# Autodesk Inventor assembly: Chassis assembly 28 Jan
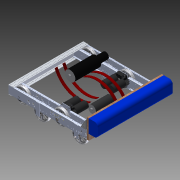
[picture p0: Inventor's stored thumbnail of the model, 180x180]
Saved by Autodesk Inventor 2014 (Build 180170000, 170)
## iProperties
Created: 2016-01-19
Part Number: Chassis assembly 28 Jan
Document SubType Name: Assembly
Designer: choices
Author: choices
## Documents named in this file (21)
- C:\Users\glasera\AppData\Local\Autodesk\Autodesk Sync\Cloud\ulanday.ian@gmail.com\2016 Robot CAD Files\ROBOT\CHASSIS\Chassis assembly 28 Jan.iam
- C:\Users\glasera\AppData\Local\Autodesk\Autodesk Sync\Cloud\ulanday.ian@gmail.com\2016 Robot CAD Files\AndyMark Chassis things\6 HiGrip with hub and double pulley.iam
- C:\Users\glasera\AppData\Local\Autodesk\Autodesk Sync\Cloud\ulanday.ian@gmail.com\2016 Robot CAD Files\AndyMark Chassis things\FR8ZZ Hex Bearing.ipt
- C:\Users\glasera\AppData\Local\Autodesk\Autodesk Sync\Cloud\ulanday.ian@gmail.com\2016 Robot CAD Files\AndyMark Chassis things\am-2598_107 2016 KOP Toughbox Mini.iam
- C:\Users\glasera\AppData\Local\Autodesk\Autodesk Sync\Cloud\ulanday.ian@gmail.com\2016 Robot CAD Files\AndyMark Chassis things\6 HiGrip with bearings, pulleys and spacers.iam
- C:\Users\glasera\AppData\Local\Autodesk\Autodesk Sync\Cloud\ulanday.ian@gmail.com\2016 Robot CAD Files\ROBOT\CHASSIS\Chass_InsideSheetTabs.ipt
- C:\Users\glasera\AppData\Local\Autodesk\Autodesk Sync\Cloud\ulanday.ian@gmail.com\2016 Robot CAD Files\AndyMark Chassis things\375-16 x 4.25 Hex Bolt_HFBOLT 0.375-16x2.5x1-C.ipt
- C:\Users\glasera\AppData\Local\Autodesk\Autodesk Sync\Cloud\ulanday.ian@gmail.com\2016 Robot CAD Files\ROBOT\CHASSIS\Chassis_OutsideSheetCustom.ipt
- C:\Users\glasera\AppData\Local\Autodesk\Autodesk Sync\Cloud\ulanday.ian@gmail.com\2016 Robot CAD Files\ROBOT\CHASSIS\Chassis_OutsideSheetCustomLeft.ipt
- C:\Users\glasera\AppData\Local\Autodesk\Autodesk Sync\Cloud\ulanday.ian@gmail.com\2016 Robot CAD Files\ROBOT\CHASSIS\Chass_InsideSheetTabsLeft.ipt
- C:\Users\glasera\AppData\Local\Autodesk\Autodesk Sync\Cloud\ulanday.ian@gmail.com\2016 Robot CAD Files\ROBOT\CHASSIS\Chass_EndCaps.ipt
- C:\Users\glasera\AppData\Local\Autodesk\Autodesk Sync\Cloud\ulanday.ian@gmail.com\2016 Robot CAD Files\ROBOT\CHASSIS\Chass_EndSheet.ipt
- C:\Users\glasera\AppData\Local\Autodesk\Autodesk Sync\Cloud\ulanday.ian@gmail.com\2016 Robot CAD Files\ROBOT\CHASSIS\Chassis_BumpermountWoodpiece.ipt
- C:\Users\glasera\AppData\Local\Autodesk\Autodesk Sync\Cloud\ulanday.ian@gmail.com\2016 Robot CAD Files\ROBOT\CHASSIS\Chassis_Bumper(29in).ipt
- C:\Users\glasera\AppData\Local\Autodesk\Autodesk Sync\Cloud\ulanday.ian@gmail.com\2016 Robot CAD Files\ROBOT\CHASSIS\Chassis_Motor.ipt
- C:\Users\glasera\AppData\Local\Autodesk\Autodesk Sync\Cloud\ulanday.ian@gmail.com\2016 Robot CAD Files\ROBOT\CHASSIS\Chassis_BumperAttachmentLeft.ipt
- C:\Users\glasera\AppData\Local\Autodesk\Autodesk Sync\Cloud\ulanday.ian@gmail.com\2016 Robot CAD Files\ROBOT\CHASSIS\Chassis_BumperAttachmentRight.ipt
- C:\Users\glasera\AppData\Local\Autodesk\Autodesk Sync\Cloud\ulanday.ian@gmail.com\2016 Robot CAD Files\ROBOT\Shooting Mechanism\Shooter_MotorTop.ipt
- C:\Users\glasera\AppData\Local\Autodesk\Autodesk Sync\Cloud\ulanday.ian@gmail.com\2016 Robot CAD Files\ROBOT\CHASSIS\Shooter_LowerMotor.ipt
- C:\Users\glasera\AppData\Local\Autodesk\Autodesk Sync\Cloud\ulanday.ian@gmail.com\2016 Robot CAD Files\ROBOT\Shooting Mechanism\Shooter_LoadingRail.ipt
- C:\Users\glasera\AppData\Local\Autodesk\Autodesk Sync\Cloud\ulanday.ian@gmail.com\2016 Robot CAD Files\ROBOT\Shooting Mechanism\Shooter_ShootingRail.ipt
## Components (35 placed, 20 different names)
1. 6 HiGrip with hub and double pulley:1 [sub-assembly] — Mate:7, Mate:8, Mate:9
2. am-2598_107 2016 KOP Toughbox Mini:1 [sub-assembly] — Mate:8, Mate:9, Mate:12, Mate:14, Flush:1, Mate:15, Mate:16, Mate:17, Insert:19, Insert:20
3. FR8ZZ Hex Bearing:1 — Mate:7, Mate:12, Mate:14, Flush:1, Mate:18, Mate:19
4. 6 HiGrip with bearings, pulleys and spacers:1 [sub-assembly] — Insert:5, Tangent:1
5. Chass_InsideSheetTabs:1 — Mate:15, Mate:16, Mate:17, Insert:5, Insert:6, Insert:8, Flush:2
6. 6 HiGrip with bearings, pulleys and spacers:2 [sub-assembly] — Insert:6
7. 6 HiGrip with bearings, pulleys and spacers:4 [sub-assembly] — Insert:8
8. Chassis_OutsideSheetCustom:1 — Mate:18, Mate:19, Insert:9, Flush:3, Mate:29, Mate:30, Flush:5, Mate:31, Mate:32, Flush:6, Angle:1, Mate:47, Mate:49
9. 375-16 x 4.25 Hex Bolt_HFBOLT 0.375-16x2.5x1-C:1 — Insert:9, Tangent:1
10. Chassis_OutsideSheetCustomLeft:1 — Insert:12, Insert:13, Insert:15, Flush:3, Mate:27, Mate:28, Flush:4, Flush:7, Flush:8, Angle:2, Angle:3
11. Chass_InsideSheetTabsLeft:1 — Mate:26, Insert:10, Insert:11, Insert:14, Insert:16, Flush:2
12. 6 HiGrip with hub and double pulley:2 [sub-assembly] — Mate:20, Mate:21, Mate:22, Mate:23
13. 6 HiGrip with bearings, pulleys and spacers:5 [sub-assembly] — Insert:13, Tangent:2
14. 6 HiGrip with bearings, pulleys and spacers:6 [sub-assembly] — Insert:15
15. 6 HiGrip with bearings, pulleys and spacers:7 [sub-assembly] — Insert:16
16. am-2598_107 2016 KOP Toughbox Mini:2 [sub-assembly] — Mate:20, Mate:21, Mate:22, Mate:24, Mate:25, Mate:26, Insert:10, Insert:11, Insert:17, Insert:18
17. FR8ZZ Hex Bearing:2 — Mate:23, Mate:24, Mate:25, Insert:12
18. 375-16 x 4.25 Hex Bolt_HFBOLT 0.375-16x2.5x1-C:2 — Insert:14, Tangent:2
19. Chass_EndCaps:1 — Mate:29, Mate:30, Flush:5, Insert:21
20. Chass_EndCaps:2 — Mate:27, Mate:28, Flush:4, Mate:33, Flush:9, Insert:22
21. Chass_EndSheet:1 — Mate:31, Mate:32, Flush:6, Flush:7
22. Chassis_BumpermountWoodpiece:1 — Mate:33, Flush:8, Flush:9, Mate:34, Flush:10, Flush:11, Mate:46
23. Chassis_Bumper(29in):1 — Mate:34, Flush:10, Flush:11
24. Chassis_Motor:1 — Insert:17
25. Chassis_Motor:2 — Insert:20
26. Chassis_Motor:3 — Insert:18, Mate:37
27. Chassis_Motor:4 — Insert:19
28. Chassis_BumperAttachmentLeft:1 — Insert:21, Angle:1
29. Chassis_BumperAttachmentRight:1 — Insert:22, Angle:2
30. Shooter_MotorTop:1 — Angle:3, Mate:37, Mate:48, Mate:49, Flush:13, Mate:50, Flush:16
31. Shooter_LowerMotor:1 — Mate:43, Mate:44, Mate:46, Mate:47, Mate:48, Flush:13
32. Shooter_LoadingRail:1 — Mate:43, Mate:45, Flush:12
33. Shooter_LoadingRail:2 — Mate:44, Mate:45, Flush:12, Flush:15
34. Shooter_ShootingRail:1 — Insert:23, Flush:14, Flush:15, Flush:16
35. Shooter_ShootingRail:2 — Insert:23, Flush:14, Mate:50
## Relationships (73: Mate 34, Insert 18, Flush 16, Angle 3, Tangent 2)
- Mate:7: 6 HiGrip with hub and double pulley:1 ↔ FR8ZZ Hex Bearing:1
- Mate:8: 6 HiGrip with hub and double pulley:1 ↔ am-2598_107 2016 KOP Toughbox Mini:1
- Mate:9: 6 HiGrip with hub and double pulley:1 ↔ am-2598_107 2016 KOP Toughbox Mini:1
- Mate:12: am-2598_107 2016 KOP Toughbox Mini:1 ↔ FR8ZZ Hex Bearing:1
- Mate:14: am-2598_107 2016 KOP Toughbox Mini:1 ↔ FR8ZZ Hex Bearing:1
- Flush:1: am-2598_107 2016 KOP Toughbox Mini:1 ↔ FR8ZZ Hex Bearing:1
- Mate:15: am-2598_107 2016 KOP Toughbox Mini:1 ↔ Chass_InsideSheetTabs:1
- Mate:16: am-2598_107 2016 KOP Toughbox Mini:1 ↔ Chass_InsideSheetTabs:1
- Mate:17: am-2598_107 2016 KOP Toughbox Mini:1 ↔ Chass_InsideSheetTabs:1
- Insert:5: 6 HiGrip with bearings, pulleys and spacers:1 ↔ Chass_InsideSheetTabs:1
- Insert:6: Chass_InsideSheetTabs:1 ↔ 6 HiGrip with bearings, pulleys and spacers:2
- Insert:8: Chass_InsideSheetTabs:1 ↔ 6 HiGrip with bearings, pulleys and spacers:4
- Mate:18: FR8ZZ Hex Bearing:1 ↔ Chassis_OutsideSheetCustom:1
- Mate:19: FR8ZZ Hex Bearing:1 ↔ Chassis_OutsideSheetCustom:1
- Insert:9: Chassis_OutsideSheetCustom:1 ↔ 375-16 x 4.25 Hex Bolt_HFBOLT 0.375-16x2.5x1-C:1
- Tangent:1: 6 HiGrip with bearings, pulleys and spacers:1 ↔ 375-16 x 4.25 Hex Bolt_HFBOLT 0.375-16x2.5x1-C:1
- Mate:20: 6 HiGrip with hub and double pulley:2 ↔ am-2598_107 2016 KOP Toughbox Mini:2
- Mate:21: 6 HiGrip with hub and double pulley:2 ↔ am-2598_107 2016 KOP Toughbox Mini:2
- Mate:22: 6 HiGrip with hub and double pulley:2 ↔ am-2598_107 2016 KOP Toughbox Mini:2
- Mate:23: 6 HiGrip with hub and double pulley:2 ↔ FR8ZZ Hex Bearing:2
- Mate:24: am-2598_107 2016 KOP Toughbox Mini:2 ↔ FR8ZZ Hex Bearing:2
- Mate:25: am-2598_107 2016 KOP Toughbox Mini:2 ↔ FR8ZZ Hex Bearing:2
- Mate:26: Chass_InsideSheetTabsLeft:1 ↔ am-2598_107 2016 KOP Toughbox Mini:2
- Insert:10: Chass_InsideSheetTabsLeft:1 ↔ am-2598_107 2016 KOP Toughbox Mini:2
- Insert:11: Chass_InsideSheetTabsLeft:1 ↔ am-2598_107 2016 KOP Toughbox Mini:2
- Insert:12: Chassis_OutsideSheetCustomLeft:1 ↔ FR8ZZ Hex Bearing:2
- Insert:13: Chassis_OutsideSheetCustomLeft:1 ↔ 6 HiGrip with bearings, pulleys and spacers:5
- Insert:14: Chass_InsideSheetTabsLeft:1 ↔ 375-16 x 4.25 Hex Bolt_HFBOLT 0.375-16x2.5x1-C:2
- Tangent:2: 6 HiGrip with bearings, pulleys and spacers:5 ↔ 375-16 x 4.25 Hex Bolt_HFBOLT 0.375-16x2.5x1-C:2
- Insert:15: Chassis_OutsideSheetCustomLeft:1 ↔ 6 HiGrip with bearings, pulleys and spacers:6
- Insert:16: Chass_InsideSheetTabsLeft:1 ↔ 6 HiGrip with bearings, pulleys and spacers:7
- Flush:2: Chass_InsideSheetTabs:1 ↔ Chass_InsideSheetTabsLeft:1
- Flush:3: Chassis_OutsideSheetCustom:1 ↔ Chassis_OutsideSheetCustomLeft:1
- Mate:27: Chassis_OutsideSheetCustomLeft:1 ↔ Chass_EndCaps:2
- Mate:28: Chassis_OutsideSheetCustomLeft:1 ↔ Chass_EndCaps:2
- Flush:4: Chassis_OutsideSheetCustomLeft:1 ↔ Chass_EndCaps:2
- Mate:29: Chassis_OutsideSheetCustom:1 ↔ Chass_EndCaps:1
- Mate:30: Chassis_OutsideSheetCustom:1 ↔ Chass_EndCaps:1
- Flush:5: Chassis_OutsideSheetCustom:1 ↔ Chass_EndCaps:1
- Mate:31: Chassis_OutsideSheetCustom:1 ↔ Chass_EndSheet:1
- Mate:32: Chassis_OutsideSheetCustom:1 ↔ Chass_EndSheet:1
- Flush:6: Chassis_OutsideSheetCustom:1 ↔ Chass_EndSheet:1
- Flush:7: Chassis_OutsideSheetCustomLeft:1 ↔ Chass_EndSheet:1
- Mate:33: Chass_EndCaps:2 ↔ Chassis_BumpermountWoodpiece:1
- Flush:8: Chassis_OutsideSheetCustomLeft:1 ↔ Chassis_BumpermountWoodpiece:1
- Flush:9: Chass_EndCaps:2 ↔ Chassis_BumpermountWoodpiece:1
- Mate:34: Chassis_BumpermountWoodpiece:1 ↔ Chassis_Bumper(29in):1
- Flush:10: Chassis_BumpermountWoodpiece:1 ↔ Chassis_Bumper(29in):1
- Flush:11: Chassis_BumpermountWoodpiece:1 ↔ Chassis_Bumper(29in):1
- Insert:17: am-2598_107 2016 KOP Toughbox Mini:2 ↔ Chassis_Motor:1
- Insert:18: am-2598_107 2016 KOP Toughbox Mini:2 ↔ Chassis_Motor:3
- Insert:19: am-2598_107 2016 KOP Toughbox Mini:1 ↔ Chassis_Motor:4
- Insert:20: am-2598_107 2016 KOP Toughbox Mini:1 ↔ Chassis_Motor:2
- Insert:21: Chass_EndCaps:1 ↔ Chassis_BumperAttachmentLeft:1
- Angle:1 (0 deg): Chassis_OutsideSheetCustom:1 ↔ Chassis_BumperAttachmentLeft:1
- Insert:22: Chass_EndCaps:2 ↔ Chassis_BumperAttachmentRight:1
- Angle:2 (0 deg): Chassis_OutsideSheetCustomLeft:1 ↔ Chassis_BumperAttachmentRight:1
- Angle:3 (0 deg): Chassis_OutsideSheetCustomLeft:1 ↔ Shooter_MotorTop:1
- Mate:37: Chassis_Motor:3 ↔ Shooter_MotorTop:1
- Mate:43: Shooter_LowerMotor:1 ↔ Shooter_LoadingRail:1
- Mate:44: Shooter_LowerMotor:1 ↔ Shooter_LoadingRail:2
- Mate:45 (50.8 mm): Shooter_LoadingRail:1 ↔ Shooter_LoadingRail:2
- Flush:12: Shooter_LoadingRail:1 ↔ Shooter_LoadingRail:2
- Mate:46 (228.6 mm): Chassis_BumpermountWoodpiece:1 ↔ Shooter_LowerMotor:1
- Mate:47: Chassis_OutsideSheetCustom:1 ↔ Shooter_LowerMotor:1
- Mate:48 (279.4 mm): Shooter_MotorTop:1 ↔ Shooter_LowerMotor:1
- Mate:49 (-215.9 mm): Chassis_OutsideSheetCustom:1 ↔ Shooter_MotorTop:1
- Flush:13 (38.1 mm): Shooter_MotorTop:1 ↔ Shooter_LowerMotor:1
- Insert:23 (50.8 mm): Shooter_ShootingRail:1 ↔ Shooter_ShootingRail:2
- Flush:14: Shooter_ShootingRail:1 ↔ Shooter_ShootingRail:2
- Mate:50: Shooter_MotorTop:1 ↔ Shooter_ShootingRail:2
- Flush:15: Shooter_LoadingRail:2 ↔ Shooter_ShootingRail:1
- Flush:16 (-76.2 mm): Shooter_MotorTop:1 ↔ Shooter_ShootingRail:1
